# Autodesk Inventor assembly: UBG-Rad
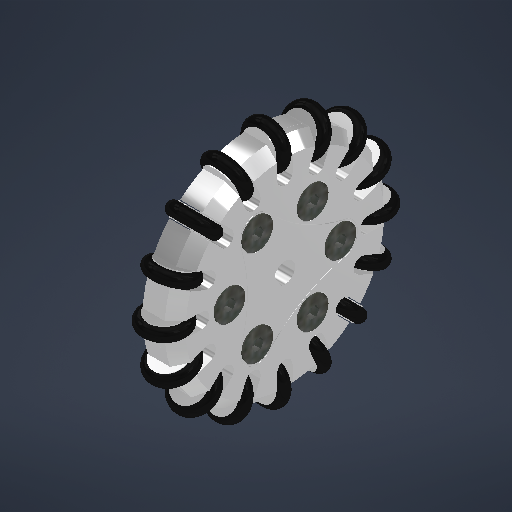
[picture p0: Inventor's stored thumbnail of the model, 512x512]
Saved by Autodesk Inventor 2025.2 (Build 292293000, 293)
## iProperties
Created: 2025-03-27
Part Number: UBG-Rad
Document SubType Name: Assembly
Designer: Faabs
Author: Faabs
## Documents named in this file (8)
- C:\Users\Faabs\Desktop\TeamFaabs-CAD v2023\UBG\Rad\UBG-Rad.iam
- C:\Users\Faabs\Desktop\TeamFaabs-CAD v2023\UBG\Rad\Radkasten.ipt
- C:\Users\Faabs\Desktop\TeamFaabs-CAD v2023\UBG\Rad\Raddeckel.ipt
- C:\Users\Faabs\Desktop\TeamFaabs-CAD v2023\UBG\Rad\Radadapter.ipt
- C:\Users\Faabs\Desktop\TeamFaabs-CAD v2023\UBG\Rad\Rolle.ipt
- C:\Users\Faabs\Desktop\TeamFaabs-CAD v2023\Verbindungselemente\Inventor\DIN 7991\DIN 7991 - M3x8.ipt
- C:\Users\Faabs\Desktop\TeamFaabs-CAD v2023\Verbindungselemente\Inventor\ISO 4032\ISO 4032 - M3.ipt
- C:\Users\Faabs\Desktop\TeamFaabs-CAD v2023\Verbindungselemente\Inventor\DIN 912\DIN 912 - M2 x 0,4 x 6 x 5.ipt
## Components (32 placed, 7 different names)
1. Radkasten:1 — Passend:1, Fluchtend:1, Passend:2, Passend:3, Passend:4, Passend:5, Passend:6, Passend:7, Passend:8, Passend:10, Passend:11, Passend:12, Passend:13, Passend:14, Passend:15, Passend:16, Passend:17
2. Raddeckel:1 — Passend:3, Passend:4, Passend:5, Passend:6, Passend:9, Einfügen:1, Einfügen:3, Einfügen:5
3. Radadapter:1 — Passend:7, Passend:8, Passend:9, Einfügen:2, Einfügen:4, Einfügen:6, Passend:24, Fluchtend:2
4. Rolle:1 — Passend:10, Passend:11
5. Rolle:2
6. Rolle:3
7. Rolle:4
8. Rolle:5
9. Rolle:6
10. Rolle:7
11. Rolle:8
12. Rolle:9
13. Rolle:10
14. Rolle:11
15. Rolle:12
16. Rolle:13
17. Rolle:14
18. Rolle:15
19. Rolle:16
20. DIN EN ISO 4032 M3:1 — Passend:17, Passend:21
21. DIN EN ISO 4032 M3:2 — Passend:16, Passend:20
22. DIN EN ISO 4032 M3:3 — Passend:12, Passend:22
23. DIN EN ISO 4032 M3:4 — Passend:15, Passend:19
24. DIN EN ISO 4032 M3:5 — Passend:13, Passend:23
25. DIN EN ISO 4032 M3:6 — Passend:14, Passend:18
26. DIN 7991 M3x8:1 — Einfügen:1, Passend:18
27. DIN 7991 M3x8:2 — Einfügen:2, Passend:19
28. DIN 7991 M3x8:3 — Einfügen:3, Passend:20
29. DIN 7991 M3x8:4 — Einfügen:4, Passend:21
30. DIN 7991 M3x8:5 — Einfügen:5, Passend:22
31. DIN 7991 M3x8:6 — Einfügen:6, Passend:23
32. DIN 912 - ersetzt durch DIN EN ISO 4762 M2 x 6:1 — Passend:24, Fluchtend:2
## Component patterns: (16 elements, first: Rolle:1)
## Relationships (32: Mate 24, Insert 6, Flush 2)
- Passend:1 [Mate]: Radkasten:1
- Fluchtend:1 [Flush]: Radkasten:1
- Passend:2 [Mate]: Radkasten:1
- Passend:3 [Mate]: Radkasten:1 ↔ Raddeckel:1
- Passend:4 [Mate]: Radkasten:1 ↔ Raddeckel:1
- Passend:5 [Mate]: Radkasten:1 ↔ Raddeckel:1
- Passend:6 [Mate]: Radkasten:1 ↔ Raddeckel:1
- Passend:7 [Mate]: Radkasten:1 ↔ Radadapter:1
- Passend:8 [Mate]: Radkasten:1 ↔ Radadapter:1
- Passend:9 [Mate]: Raddeckel:1 ↔ Radadapter:1
- Passend:10 [Mate]: Radkasten:1 ↔ Rolle:1
- Passend:11 [Mate] (0.125 mm): Radkasten:1 ↔ Rolle:1
- Einfügen:1 [Insert]: Raddeckel:1 ↔ DIN 7991 M3x8:1
- Einfügen:2 [Insert]: Radadapter:1 ↔ DIN 7991 M3x8:2
- Einfügen:3 [Insert]: Raddeckel:1 ↔ DIN 7991 M3x8:3
- Einfügen:4 [Insert]: Radadapter:1 ↔ DIN 7991 M3x8:4
- Einfügen:5 [Insert]: Raddeckel:1 ↔ DIN 7991 M3x8:5
- Einfügen:6 [Insert]: Radadapter:1 ↔ DIN 7991 M3x8:6
- Passend:12 [Mate]: Radkasten:1 ↔ DIN EN ISO 4032 M3:3
- Passend:13 [Mate]: Radkasten:1 ↔ DIN EN ISO 4032 M3:5
- Passend:14 [Mate]: Radkasten:1 ↔ DIN EN ISO 4032 M3:6
- Passend:15 [Mate]: Radkasten:1 ↔ DIN EN ISO 4032 M3:4
- Passend:16 [Mate]: Radkasten:1 ↔ DIN EN ISO 4032 M3:2
- Passend:17 [Mate]: Radkasten:1 ↔ DIN EN ISO 4032 M3:1
- Passend:18 [Mate]: DIN EN ISO 4032 M3:6 ↔ DIN 7991 M3x8:1
- Passend:19 [Mate]: DIN EN ISO 4032 M3:4 ↔ DIN 7991 M3x8:2
- Passend:20 [Mate]: DIN EN ISO 4032 M3:2 ↔ DIN 7991 M3x8:3
- Passend:21 [Mate]: DIN EN ISO 4032 M3:1 ↔ DIN 7991 M3x8:4
- Passend:22 [Mate]: DIN EN ISO 4032 M3:3 ↔ DIN 7991 M3x8:5
- Passend:23 [Mate]: DIN EN ISO 4032 M3:5 ↔ DIN 7991 M3x8:6
- Passend:24 [Mate]: Radadapter:1 ↔ DIN 912 - ersetzt durch DIN EN ISO 4762 M2 x 6:1
- Fluchtend:2 [Flush]: Radadapter:1 ↔ DIN 912 - ersetzt durch DIN EN ISO 4762 M2 x 6:1
